# Autodesk Inventor assembly: Recessed Wheels V1.0
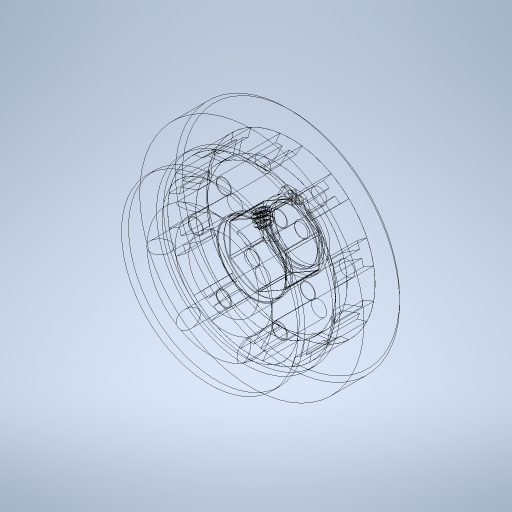
[picture p0: Inventor's stored thumbnail of the model, 512x512]
Saved by Autodesk Inventor 2023.2 (Build 272271000, 271)
## iProperties
Created: 2023-02-06
Part Number: Recessed Wheels V1.0
Document SubType Name: Assembly
Designer: Nathan Cai
Mass: 29.776 g
Surface Area: 113.605 cm^2
Volume: 23.0692 cm^3
Author: Nathan Cai
## Documents named in this file (5)
- E:\Documents\Inventor\Chort V2.0\Custom Wheel V2.0\Recessed Wheels V2.0.iam
- E:\Documents\Inventor\Chort V2.0\Custom Wheel V2.0\Tire Hub.ipt
- E:\Documents\Inventor\Chort V2.0\Custom Wheel V2.0\Tire.ipt
- E:\Documents\Inventor\Chort V2.0\Custom Wheel V2.0\T40_Hub_With_Retainer\T40_Hub_With_Retainer.iam
- E:\Documents\Inventor\Chort V2.0\Pulley.ipt
## Components (4 placed, 4 different names)
1. Tire Hub:1 — Flush:5, Mate:5, Mate:6, Mate:7, Flush:6, Mate:9, Mate:10
2. Tire:1 — Flush:5, Mate:5, Mate:8
3. T40_Hub_With_Retainer:1 [sub-assembly] — Mate:6, Mate:7, Flush:6
4. Pulley:1 — Mate:8, Mate:9, Mate:10
## Relationships (8: Mate 6, Flush 2)
- Flush:5: Tire Hub:1 ↔ Tire:1
- Mate:5: Tire Hub:1 ↔ Tire:1
- Mate:6: Tire Hub:1 ↔ T40_Hub_With_Retainer:1
- Mate:7 (0.0635 mm): Tire Hub:1 ↔ T40_Hub_With_Retainer:1
- Flush:6: Tire Hub:1 ↔ T40_Hub_With_Retainer:1
- Mate:8: Tire:1 ↔ Pulley:1
- Mate:9: Tire Hub:1 ↔ Pulley:1
- Mate:10: Tire Hub:1 ↔ Pulley:1
